# Autodesk Inventor assembly: batt support
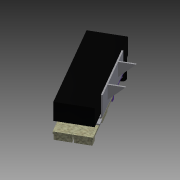
[picture p0: Inventor's stored thumbnail of the model, 180x180]
Saved by Autodesk Inventor 2015 (Build 190159000, 159)
## iProperties
Created: 2015-05-04
Part Number: batt support
Document SubType Name: Assembly
Designer: Kuba
Author: Kuba
## Documents named in this file (10)
- C:\Users\Kuba\Dysk Google\synergia\Synergolf\model\GOLF\batt support\batt support.iam
- C:\Users\Kuba\Dysk Google\synergia\Synergolf\model\GOLF\lipol_6000.ipt
- C:\Users\Kuba\Dysk Google\synergia\Synergolf\model\GOLF\batt support\dociskacz.ipt
- C:\Users\Kuba\Dysk Google\synergia\Synergolf\model\GOLF\batt support\batt-logic support.ipt
- C:\Users\Kuba\Dysk Google\synergia\Synergolf\model\GOLF\rbc support\rbc support.iam
- C:\Users\Kuba\Dysk Google\synergia\Synergolf\model\GOLF\batt support\step up.ipt
- C:\Users\Kuba\Dysk Google\synergia\Synergolf\model\GOLF\batt support\step down.ipt
- C:\Users\Kuba\Dysk Google\synergia\Synergolf\model\GOLF\ContentCenter\pl-PL\DIN 912\DIN 912 - M3 x 0,5 x 12 x 10,75.ipt
- C:\Users\Kuba\Dysk Google\synergia\Synergolf\model\GOLF\batt support\dystans rbc.ipt
- C:\Users\Kuba\Dysk Google\synergia\Synergolf\model\GOLF\driver\wspornik.ipt
## Components (17 placed, 9 different names)
1. lipol_6000:1 — Równoległy:1, Zestawiający:1, Zestawiający:2, Zestawiający:3, Równoległy:2, Zestawiający:4, Równoległy:8
2. batt-logic support:1 — Zestawiający:3, Równoległy:2, Zestawiający:4, Równoległy:7, Zestawiający:8, Równoległy:13, Równoległy:14, Zestawiający:9, Równoległy:15, Równoległy:16
3. rbc support:1 [sub-assembly] — Równoległy:5, Zestawiający:6, Równoległy:6, Równoległy:7, Równoległy:8
4. step up:1 — Wstaw:1, Wstaw:2, Wstaw:11, Wstaw:12, Zestawiający:5, Równoległy:4, Równoległy:6
5. step down:1 — Wstaw:3, Wstaw:4, Wstaw:13, Wstaw:14, Zestawiający:5, Równoległy:4, Zestawiający:6
6. DIN 912 - zastąpiona przez DIN EN ISO 4762 M3 x 12:3 — Wstaw:1
7. DIN 912 - zastąpiona przez DIN EN ISO 4762 M3 x 12:4 — Wstaw:2
8. DIN 912 - zastąpiona przez DIN EN ISO 4762 M3 x 12:1 — Wstaw:3
9. DIN 912 - zastąpiona przez DIN EN ISO 4762 M3 x 12:2 — Wstaw:4
10. dystans rbc:1 — Wstaw:11
11. dystans rbc:2 — Wstaw:12, Równoległy:3
12. dystans rbc:3 — Wstaw:13, Równoległy:3, Równoległy:5
13. dystans rbc:4 — Wstaw:14
14. wspornik:1 — Zestawiający:9, Równoległy:15, Równoległy:16
15. wspornik:2 — Zestawiający:8, Równoległy:13, Równoległy:14
16. dociskacz:1 — Równoległy:1, Zestawiający:1, Zestawiający:2
17. dociskacz:2
## Component patterns: (2 elements, first: dociskacz:1)
## Relationships (28: Flush 12, Mate 8, Insert 8)
- Równoległy:1 [Flush]: lipol_6000:1 ↔ dociskacz:1
- Zestawiający:1 [Mate]: lipol_6000:1 ↔ dociskacz:1
- Zestawiający:2 [Mate] (-30 mm): lipol_6000:1 ↔ dociskacz:1
- Zestawiający:3 [Mate]: lipol_6000:1 ↔ batt-logic support:1
- Równoległy:2 [Flush]: lipol_6000:1 ↔ batt-logic support:1
- Zestawiający:4 [Mate]: lipol_6000:1 ↔ batt-logic support:1
- Wstaw:1 [Insert]: step up:1 ↔ DIN 912 - zastąpiona przez DIN EN ISO 4762 M3 x 12:3
- Wstaw:2 [Insert]: step up:1 ↔ DIN 912 - zastąpiona przez DIN EN ISO 4762 M3 x 12:4
- Wstaw:3 [Insert]: step down:1 ↔ DIN 912 - zastąpiona przez DIN EN ISO 4762 M3 x 12:1
- Wstaw:4 [Insert]: step down:1 ↔ DIN 912 - zastąpiona przez DIN EN ISO 4762 M3 x 12:2
- Wstaw:11 [Insert]: step up:1 ↔ dystans rbc:1
- Wstaw:12 [Insert]: step up:1 ↔ dystans rbc:2
- Wstaw:13 [Insert]: step down:1 ↔ dystans rbc:3
- Wstaw:14 [Insert]: step down:1 ↔ dystans rbc:4
- Równoległy:3 [Flush]: dystans rbc:2 ↔ dystans rbc:3
- Zestawiający:5 [Mate] (3 mm): step up:1 ↔ step down:1
- Równoległy:4 [Flush]: step up:1 ↔ step down:1
- Równoległy:5 [Flush]: rbc support:1 ↔ dystans rbc:3
- Zestawiający:6 [Mate] (3 mm): rbc support:1 ↔ step down:1
- Równoległy:6 [Flush]: rbc support:1 ↔ step up:1
- Równoległy:7 [Flush]: batt-logic support:1 ↔ rbc support:1
- Równoległy:8 [Flush] (-3 mm): lipol_6000:1 ↔ rbc support:1
- Zestawiający:8 [Mate]: batt-logic support:1 ↔ wspornik:2
- Równoległy:13 [Flush]: batt-logic support:1 ↔ wspornik:2
- Równoległy:14 [Flush] (20 mm): batt-logic support:1 ↔ wspornik:2
- Zestawiający:9 [Mate]: batt-logic support:1 ↔ wspornik:1
- Równoległy:15 [Flush]: batt-logic support:1 ↔ wspornik:1
- Równoległy:16 [Flush] (20 mm): batt-logic support:1 ↔ wspornik:1
